# Autodesk Inventor assembly: Дифференциал
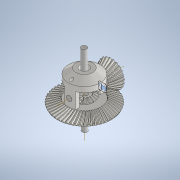
[picture p0: Inventor's stored thumbnail of the model, 180x180]
Saved by Autodesk Inventor 2020 (Build 240168000, 168)
## iProperties
Created: 2021-02-28
Part Number: Дифференциал
Document SubType Name: Assembly
Designer: Антон
Author: Антон
## Documents named in this file (6)
- D:\Project\Robots\RRO 2021\Differential\Дифференциал.iam
- D:\Project\Robots\RRO 2021\Differential\Дифференциал\Мастер проектирования\Конические зубчатые колеса1.iam
- D:\Project\Robots\RRO 2021\Differential\Ось сателлитов.ipt
- D:\Project\Robots\RRO 2021\Differential\Дифференциал\Мастер проектирования\Конические зубчатые колеса2.iam
- D:\Project\Robots\RRO 2021\Differential\Ось колес.ipt
- D:\Project\Robots\RRO 2021\Differential\Дифференциал\Мастер проектирования\Конические зубчатые колеса2_КОПИЯ1.iam
## Components (6 placed, 5 different names)
1. Основа дифференциала [sub-assembly] — С поворотом:1, Совмещение:1, Угол:1
2. Ось сателлитов:1 — С поворотом:1, С поворотом:2, С поворотом:3
3. Сателлит левый [sub-assembly] — С поворотом:2, Жесткий:1
4. Выходная ось:1 — Жесткий:1
5. Выходная ось:2 — Жесткий:2
6. Конические зубчатые колеса2_КОПИЯ1:1 [sub-assembly] — С поворотом:3, Жесткий:2
## Relationships (7: RevoluteJoint 3, WeldJoint 2, Mate 1, Angle 1)
- С поворотом:1 [RevoluteJoint]: Основа дифференциала ↔ Ось сателлитов:1
- С поворотом:2 [RevoluteJoint] (-5 mm): Ось сателлитов:1 ↔ Сателлит левый
- Совмещение:1 [Mate]: Основа дифференциала
- Угол:1 [Angle] (0 deg): Основа дифференциала
- Жесткий:1 [WeldJoint]: Сателлит левый ↔ Выходная ось:1
- С поворотом:3 [RevoluteJoint] (-5 mm): Ось сателлитов:1 ↔ Конические зубчатые колеса2_КОПИЯ1:1
- Жесткий:2 [WeldJoint]: Выходная ось:2 ↔ Конические зубчатые колеса2_КОПИЯ1:1
